# Autodesk Inventor assembly: 4.L - GM - 01.00
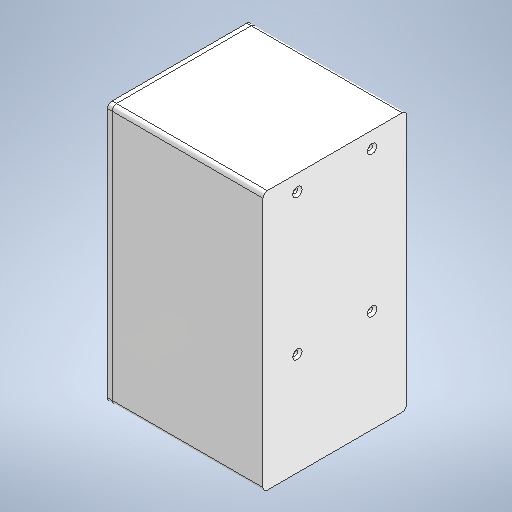
[picture p0: Inventor's stored thumbnail of the model, 512x512]
Saved by Autodesk Inventor 2025.2 (Build 292293000, 293)
## iProperties
Created: 2025-03-27
Part Number: 4.L - GM - 01.00
Document SubType Name: Assembly
Designer: hepma_axt67em
Mass: 457.202 g
Surface Area: 1871.67 cm^2
Volume: 281.182 cm^3
Density: 1.626 g/cm^3
Author: hepma_axt67em
## Documents named in this file (5)
- C:\Users\hepma_axt67em\Documents\Inventor\GeigerCounter\box.iam
- C:\Users\hepma_axt67em\Documents\Inventor\GeigerCounter\box_bottom.ipt
- C:\Users\hepma_axt67em\Documents\Inventor\GeigerCounter\box_top.ipt
- C:\Users\hepma_axt67em\Documents\Inventor\GeigerCounter\cover.ipt
- C:\Users\hepma_axt67em\Documents\Inventor\GeigerCounter\holder.ipt
## Components (4 placed, 4 different names)
1. box_bottom:1 — Proti sobě:6, Proti sobě:7, Proti sobě:8
2. box_top:1 — Proti sobě:1, Proti sobě:2, Proti sobě:3, Proti sobě:4, Proti sobě:5, Proti sobě:6, Proti sobě:7, Proti sobě:8
3. cover:1 — Proti sobě:4, Proti sobě:5, Proti sobě:9
4. holder:1 — Proti sobě:1, Proti sobě:2, Proti sobě:3
## Relationships (9: Mate 9)
- Proti sobě:1 [Mate]: box_top:1 ↔ holder:1
- Proti sobě:2 [Mate]: box_top:1 ↔ holder:1
- Proti sobě:3 [Mate]: box_top:1 ↔ holder:1
- Proti sobě:4 [Mate]: box_top:1 ↔ cover:1
- Proti sobě:5 [Mate]: box_top:1 ↔ cover:1
- Proti sobě:6 [Mate]: box_bottom:1 ↔ box_top:1
- Proti sobě:7 [Mate]: box_bottom:1 ↔ box_top:1
- Proti sobě:8 [Mate]: box_bottom:1 ↔ box_top:1
- Proti sobě:9 [Mate]: cover:1
